# Autodesk Inventor assembly: PortaMarcador
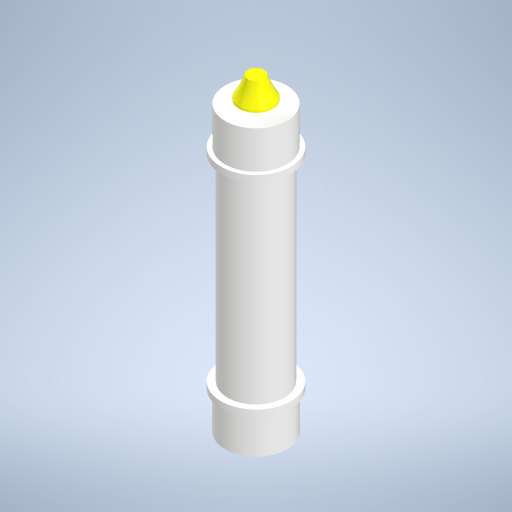
[picture p0: Inventor's stored thumbnail of the model, 512x512]
Saved by Autodesk Inventor 2023.1 (Build 271208000, 208)
## iProperties
Created: 2022-08-24
Part Number: PortaMarcador
Document SubType Name: Assembly
Designer: Daniel Peña
Author: Daniel Peña
## Documents named in this file (5)
- C:\Users\danie_p\Documents\Inventor\Lab1Robotica\PortaMarcador.iam
- C:\Users\danie_p\Documents\Inventor\Lab1Robotica\TuboMarcador.ipt
- C:\Users\danie_p\Documents\Inventor\Lab1Robotica\Marcador.ipt
- C:\Users\danie_p\Documents\Inventor\Content Center Files\R2023\en-US\DIN 8063 K\DIN 8063 Cap Type K 25.ipt
- C:\Users\danie_p\Documents\Inventor\Lab1Robotica\baseBot.ipt
## Components (5 placed, 4 different names)
1. TuboMarcador:1 — Insert:1, Insert:2, Insert:3, Tangent:1, Mate:1, Insert:4
2. Marcador:1 — Insert:1
3. DIN 8063 Cap Type K 25:1 — Insert:2
4. DIN 8063 Cap Type K 25:2 — Insert:3
5. baseBot:1 — Mate:1, Insert:4
## Relationships (6: Insert 4, Tangent 1, Mate 1)
- Insert:1 (-90 mm): TuboMarcador:1 ↔ Marcador:1
- Insert:2: TuboMarcador:1 ↔ DIN 8063 Cap Type K 25:1
- Insert:3: TuboMarcador:1 ↔ DIN 8063 Cap Type K 25:2
- Tangent:1: TuboMarcador:1
- Mate:1: TuboMarcador:1 ↔ baseBot:1
- Insert:4 (20 mm): TuboMarcador:1 ↔ baseBot:1
